# Autodesk Inventor assembly: LCD12864_Mine
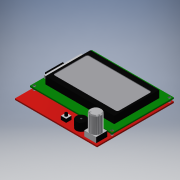
[picture p0: Inventor's stored thumbnail of the model, 180x180]
Saved by Autodesk Inventor 2016 (Build 200138000, 138)
## iProperties
Created: 2015-06-10
Part Number: LCD12864_Mine
Document SubType Name: Assembly
Designer: Mathias L. Kjeldgaard
Author: Mathias L. Kjeldgaard
## Documents named in this file (3)
- C:\Users\PowerStation9000\AppData\Local\Autodesk\Autodesk Sync\Cloud\mathiaslk\UltiBot mk2\Importerede komponenter\LCD 12864 Skærm (Stor)\LCD12864_Mine.iam
- C:\Users\PowerStation9000\AppData\Local\Autodesk\Autodesk Sync\Cloud\mathiaslk\UltiBot mk2\Importerede komponenter\LCD 12864 Skærm (Stor)\Rød PCB.ipt
- C:\Users\PowerStation9000\AppData\Local\Autodesk\Autodesk Sync\Cloud\mathiaslk\UltiBot mk2\Importerede komponenter\LCD 12864 Skærm (Stor)\Grøn PCB.ipt
## Components (2 placed, 2 different names)
1. Rød PCB:1 — Flush:1, Flush:2
2. Grøn PCB:1 — Flush:1, Flush:2
## Relationships (2: Flush 2)
- Flush:1: Rød PCB:1 ↔ Grøn PCB:1
- Flush:2 (2.54 mm): Rød PCB:1 ↔ Grøn PCB:1
